# Autodesk Inventor assembly: 220LB-ASSY
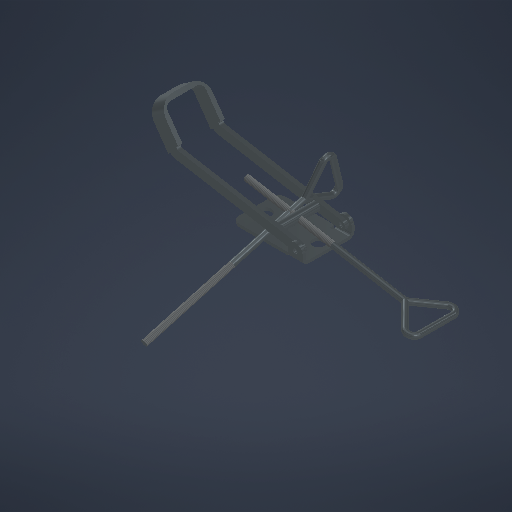
[picture p0: Inventor's stored thumbnail of the model, 512x512]
Saved by Autodesk Inventor 2025.3 (Build 293356030, 356C)
## iProperties
Created: 2025-08-31
Part Number: 220LB-ASSY
Document SubType Name: Assembly
Designer: lstk1ng
Author: lstk1ng
## Documents named in this file (5)
- C:\Users\lstk1ng\Documents\UPC\UPC-10\PROYECTO MECATRONICO 1\DISEÑO MECANICO\220LB LOCK\220LB-ASSY.iam
- C:\Users\lstk1ng\Documents\UPC\UPC-10\PROYECTO MECATRONICO 1\DISEÑO MECANICO\220LB LOCK\BODY-220LB.ipt
- C:\Users\lstk1ng\Documents\UPC\UPC-10\PROYECTO MECATRONICO 1\DISEÑO MECANICO\220LB LOCK\GRIPPER-220LB.ipt
- C:\Users\lstk1ng\Documents\UPC\UPC-10\PROYECTO MECATRONICO 1\DISEÑO MECANICO\220LB LOCK\PLATE-220.ipt
- C:\Users\lstk1ng\Documents\UPC\UPC-10\PROYECTO MECATRONICO 1\DISEÑO MECANICO\220LB LOCK\GRIPPER-220LB_MIR.ipt
## Components (4 placed, 4 different names)
1. BODY-220LB:1 — Mate:1, Insert:1, Cylindrical:1
2. GRIPPER-220LB:1 — Cylindrical:1, Mate:2, Cylindrical:2
3. PLATE-220:1 — Mate:1, Insert:1
4. GRIPPER-220LB_MIR:1 — Mate:2, Cylindrical:2
## Relationships (5: Mate 2, CylindricalJoint 2, Insert 1)
- Mate:1: BODY-220LB:1 ↔ PLATE-220:1
- Insert:1: BODY-220LB:1 ↔ PLATE-220:1
- Cylindrical:1: BODY-220LB:1 ↔ GRIPPER-220LB:1
- Mate:2: GRIPPER-220LB:1 ↔ GRIPPER-220LB_MIR:1
- Cylindrical:2: GRIPPER-220LB:1 ↔ GRIPPER-220LB_MIR:1
